# Autodesk Inventor assembly: BoyaEnsamble
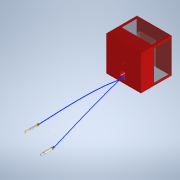
[picture p0: Inventor's stored thumbnail of the model, 180x180]
Saved by Autodesk Inventor 2020 (Build 240168000, 168)
## iProperties
Created: 2021-10-16
Part Number: BoyaEnsamble
Document SubType Name: Assembly
Designer: DANIEL
Author: DANIEL
## Documents named in this file (13)
- C:\Users\DANIEL\Documents\Personal\Convocatorias\Escollera\tesis\CAD\BoyaEnsamble.iam
- C:\Users\DANIEL\Documents\Personal\Convocatorias\Escollera\tesis\CAD\CajaBoya.ipt
- C:\Users\DANIEL\Documents\Personal\Convocatorias\Escollera\tesis\CAD\cajaEléctrica.ipt
- C:\Users\DANIEL\Documents\Personal\Convocatorias\Escollera\tesis\CAD\W520.iam
- C:\Users\DANIEL\Documents\Personal\Convocatorias\Escollera\tesis\CAD\techo.ipt
- C:\Users\DANIEL\Documents\Personal\Convocatorias\Escollera\tesis\CAD\EnsamblajeCircuito.iam
- C:\Users\DANIEL\Documents\Personal\Convocatorias\Escollera\tesis\CAD\antena.ipt
- C:\Users\DANIEL\Documents\Personal\Convocatorias\Escollera\tesis\CAD\BoyaEnsamble\AIP\Tubos y tuberías\Cable y arnés\BoyaEnsamble.Arnés2.iam
- C:\Users\DANIEL\Documents\Personal\Convocatorias\Escollera\tesis\CAD\W504.ipt
- C:\Users\DANIEL\Documents\Personal\Convocatorias\Escollera\tesis\CAD\packBaterias.iam
- C:\Users\DANIEL\Documents\Personal\Convocatorias\Escollera\tesis\CAD\BoyaEnsamble\AIP\Tubos y tuberías\Cable y arnés\BoyaEnsamble.Arnés3.iam
- C:\Users\DANIEL\Documents\Personal\Convocatorias\Escollera\tesis\CAD\BoyaEnsamble\AIP\Tubos y tuberías\Cable y arnés\BoyaEnsamble.Arnés4.iam
- C:\Users\DANIEL\Documents\Personal\Convocatorias\Escollera\tesis\CAD\panelSolar.ipt
## Components (12 placed, 12 different names)
1. CajaBoya:1 — Coincidencia:1, Coincidencia:2, Coincidencia:3, Coincidencia:4
2. cajaEléctrica:1 — Coincidencia:1, Coincidencia:2
3. W520:1 [sub-assembly] — Coincidencia:3
4. techo:1
5. EnsamblajeCircuito:1 [sub-assembly]
6. antena:1
7. Arnés2 [sub-assembly]
8. W504:1
9. packBaterias:1 [sub-assembly]
10. Arnés3 [sub-assembly]
11. Arnés4 [sub-assembly]
12. panelSolar:1 — Coincidencia:4
## Relationships (4: Mate 4)
- Coincidencia:1 [Mate]: CajaBoya:1 ↔ cajaEléctrica:1
- Coincidencia:2 [Mate]: CajaBoya:1 ↔ cajaEléctrica:1
- Coincidencia:3 [Mate] (1000 mm): CajaBoya:1 ↔ W520:1
- Coincidencia:4 [Mate]: CajaBoya:1 ↔ panelSolar:1
